# Autodesk Inventor assembly: Portable_Amp_Speaker
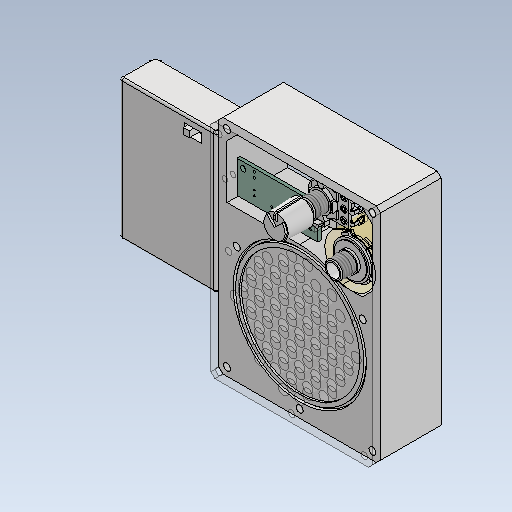
[picture p0: Inventor's stored thumbnail of the model, 512x512]
Saved by Autodesk Inventor 2026.1 (Build 301233020, 233B)
## iProperties
Created: 2026-08-13
Part Number: Portable_Amp_Speaker
Document SubType Name: Assembly
Designer: ug_nd
Author: ug_nd
## Documents named in this file (9)
- C:\Users\ug_nd\git_local\Portable_Amp_Speaker\hardware\Portable_Amp_Speaker.iam
- C:\Users\ug_nd\git_local\Portable_Amp_Speaker\hardware\speaker.ipt
- C:\Users\ug_nd\git_local\Portable_Amp_Speaker\hardware\circuit.iam
- C:\Users\ug_nd\git_local\Portable_Amp_Speaker\hardware\batt_box.ipt
- C:\Users\ug_nd\git_local\Portable_Amp_Speaker\hardware\phon_jack.ipt
- C:\Users\ug_nd\git_local\Portable_Amp_Speaker\hardware\potentiometer.ipt
- C:\Users\ug_nd\git_local\Portable_Amp_Speaker\hardware\knob.ipt
- C:\Users\ug_nd\git_local\Portable_Amp_Speaker\hardware\front_pannel.ipt
- C:\Users\ug_nd\git_local\Portable_Amp_Speaker\hardware\housing_3dp.ipt
## Components (8 placed, 8 different names)
1. speaker:1 — メイト:1, メイト:2, フラッシュ:1, フラッシュ:2, 正接:1, フラッシュ:3, フラッシュ:4
2. circuit:1 [sub-assembly] — フラッシュ:2, メイト:3, 正接:1, メイト:12, メイト:13
3. batt_box:1
4. phon_jack:1 — フラッシュ:3, メイト:11, 角度:2
5. potentiometer:1 — フラッシュ:4, 角度:1, メイト:7, メイト:8, メイト:10, 角度:3
6. knob:1 — 角度:1, メイト:7, メイト:8
7. front_pannel:1 — メイト:9, メイト:10, メイト:11, メイト:12, メイト:13, メイト:14, メイト:15, メイト:16
8. housing_3dp:1 — メイト:14, メイト:15, メイト:16
## Relationships (21: Mate 13, Flush 4, Angle 3, Tangent 1)
- メイト:1 [Mate]: speaker:1
- メイト:2 [Mate]: speaker:1
- フラッシュ:1 [Flush]: speaker:1
- フラッシュ:2 [Flush] (5 mm): speaker:1 ↔ circuit:1
- メイト:3 [Mate] (35 mm): circuit:1
- 正接:1 [Tangent] (3.25 mm): speaker:1 ↔ circuit:1
- フラッシュ:3 [Flush]: speaker:1 ↔ phon_jack:1
- フラッシュ:4 [Flush]: speaker:1 ↔ potentiometer:1
- 角度:1 [Angle] (180 deg): potentiometer:1 ↔ knob:1
- メイト:7 [Mate]: potentiometer:1 ↔ knob:1
- メイト:8 [Mate]: potentiometer:1 ↔ knob:1
- メイト:9 [Mate]: front_pannel:1
- メイト:10 [Mate]: potentiometer:1 ↔ front_pannel:1
- メイト:11 [Mate]: phon_jack:1 ↔ front_pannel:1
- メイト:12 [Mate]: circuit:1 ↔ front_pannel:1
- メイト:13 [Mate]: circuit:1 ↔ front_pannel:1
- 角度:2 [Angle] (0 deg): phon_jack:1
- 角度:3 [Angle] (0 deg): potentiometer:1
- メイト:14 [Mate]: front_pannel:1 ↔ housing_3dp:1
- メイト:15 [Mate]: front_pannel:1 ↔ housing_3dp:1
- メイト:16 [Mate]: front_pannel:1 ↔ housing_3dp:1
